# Autodesk Inventor assembly: CollectorAssembly
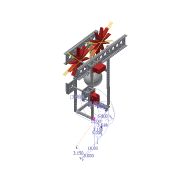
[picture p0: Inventor's stored thumbnail of the model, 180x180]
Saved by Autodesk Inventor 2018 (Build 220112000, 112)
## iProperties
Created: 2018-10-28
Part Number: CollectorAssembly
Document SubType Name: Assembly
Designer: ball
Author: ball
## Documents named in this file (18)
- C:\FTC\FTC8863CAD\2018Robot\CollectorAssembly.iam
- C:\FTC\FTC8863CAD\GoBilda\1103 Parts\1106-0035-0280.ipt
- C:\FTC\FTC8863CAD\GoBilda\1121 Parts\1121-0011-0288.ipt
- C:\FTC\FTC8863CAD\2018Robot\ServoWithPlateCoupler.iam
- C:\FTC\FTC8863CAD\GoBilda\1501 Parts\1501-0006-0240.ipt
- C:\FTC\FTC8863CAD\GoBilda\2905 Parts\2905-0006-0008 assembly.ipt
- C:\FTC\FTC8863CAD\GoBilda\1601 Parts\1601-0014-0006.ipt
- C:\FTC\FTC8863CAD\GoBilda\2101 Parts\2101-0006-0090.ipt
- C:\FTC\FTC8863CAD\Andymark\am-0619a+Entrapption+Star,+4.75+Diameter.ipt
- C:\FTC\FTC8863CAD\Andymark\am-2850+wiffle+base+Ball.ipt
- C:\FTC\FTC8863CAD\GoBilda\1103 Parts\1103-0011-0088.ipt
- C:\FTC\FTC8863CAD\GoBilda\1121 Parts\1121-0007-0192.ipt
- C:\FTC\FTC8863CAD\GoBilda\1106 Parts\1106-0010-0080.ipt
- C:\FTC\FTC8863CAD\RevRobotics\REV-31-1537.ipt
- C:\FTC\FTC8863CAD\GoBilda\1121 Parts\1121-0001-0048.ipt
- C:\FTC\FTC8863CAD\GoBilda\2101 Parts\2101-0006-0080.ipt
- C:\FTC\FTC8863CAD\GoBilda\1106 Parts\1106-0009-0072.ipt
- C:\FTC\FTC8863CAD\2018Robot\TransferChute.ipt
## Components (33 placed, 17 different names)
1. 1106-0035-0280:1 — Flush:1, Flush:2, Flush:4, Mate:62, Mate:63, Flush:5, Mate:70, Mate:101
2. 1106-0035-0280:2 — Flush:1, Flush:4, Mate:13, Mate:57, Mate:59, Mate:69, Mate:90, Mate:91, Mate:92
3. 1106-0035-0280:3 — Flush:2, Mate:58, Mate:69, Mate:74, Mate:75, Mate:93, Mate:95
4. 1106-0035-0280:4 — Mate:61, Flush:5, Mate:64, Mate:70, Mate:99, Mate:102, Mate:104
5. 1121-0011-0288:1 — Mate:13, Mate:22, Mate:23, Mate:24, Mate:25, Mate:26, Mate:27, Mate:37, Mate:38, Mate:68
6. ServoWithPlateCoupler:1 [sub-assembly] — Mate:15, Mate:17, Mate:19, Mate:21, Mate:22, Mate:27
7. 1501-0006-0240:2 — Mate:15, Mate:23
8. 1501-0006-0240:3 — Mate:19, Mate:25
9. 1501-0006-0240:4 — Mate:17, Mate:26
10. 1501-0006-0240:5 — Mate:21, Mate:24
11. 2905-0006-0008 assembly:1 — Mate:42, Mate:43
12. 2905-0006-0008 assembly:2 — Mate:44, Mate:45
13. 1601-0014-0006:1 — Mate:41, Mate:42, Mate:66
14. 1601-0014-0006:2 — Mate:37, Mate:38, Mate:40, Mate:44
15. 2101-0006-0090:1 — Mate:40, Mate:41, Mate:43, Mate:45, Mate:65, Mate:66, Mate:67
16. am-0619a+Entrapption+Star,+4.75+Diameter:1 — Mate:67, Mate:97
17. am-0619a+Entrapption+Star,+4.75+Diameter:2 — Mate:68, Mate:98
18. am-2850+wiffle+base+Ball:1
19. 1103-0011-0088:2 — Mate:61, Mate:62, Mate:63, Mate:78
20. 1103-0011-0088:3 — Mate:57, Mate:58, Mate:59, Mate:76, Mate:77, Flush:6
21. 1121-0007-0192:2 — Mate:64, Mate:65, Mate:74, Mate:75, Mate:97, Mate:98
22. 1106-0010-0080:1 — Mate:76, Mate:77, Flush:6, Mate:78
23. REV-31-1537:3 — Mate:99, Mate:103, Mate:104
24. ServoWithPlateCoupler:2 [sub-assembly] — Mate:88, Mate:89, Angle:1, Flush:8
25. 1501-0006-0240:6 — Mate:83, Mate:86
26. 1501-0006-0240:7 — Mate:84
27. 1501-0006-0240:8 — Mate:85
28. 1501-0006-0240:9 — Mate:88
29. 1121-0001-0048:1 — Mate:83, Mate:84, Mate:85, Mate:86, Mate:89, Angle:1, Mate:90, Mate:91, Mate:92, Mate:94, Flush:7
30. 1121-0001-0048:2 — Mate:93, Mate:94, Flush:7, Mate:95
31. 2101-0006-0080:2 — Flush:8
32. 1106-0009-0072:1 — Mate:101, Mate:102, Mate:103
33. TransferChute:1
## Relationships (69: Mate 61, Flush 7, Angle 1)
- Flush:1: 1106-0035-0280:1 ↔ 1106-0035-0280:2
- Flush:2: 1106-0035-0280:1 ↔ 1106-0035-0280:3
- Flush:4: 1106-0035-0280:1 ↔ 1106-0035-0280:2
- Mate:13: 1106-0035-0280:2 ↔ 1121-0011-0288:1
- Mate:15: ServoWithPlateCoupler:1 ↔ 1501-0006-0240:2
- Mate:17: ServoWithPlateCoupler:1 ↔ 1501-0006-0240:4
- Mate:19: ServoWithPlateCoupler:1 ↔ 1501-0006-0240:3
- Mate:21: ServoWithPlateCoupler:1 ↔ 1501-0006-0240:5
- Mate:22: 1121-0011-0288:1 ↔ ServoWithPlateCoupler:1
- Mate:23: 1121-0011-0288:1 ↔ 1501-0006-0240:2
- Mate:24: 1121-0011-0288:1 ↔ 1501-0006-0240:5
- Mate:25: 1121-0011-0288:1 ↔ 1501-0006-0240:3
- Mate:26: 1121-0011-0288:1 ↔ 1501-0006-0240:4
- Mate:27 (24 mm): 1121-0011-0288:1 ↔ ServoWithPlateCoupler:1
- Mate:37: 1121-0011-0288:1 ↔ 1601-0014-0006:2
- Mate:38: 1121-0011-0288:1 ↔ 1601-0014-0006:2
- Mate:40: 1601-0014-0006:2 ↔ 2101-0006-0090:1
- Mate:41: 1601-0014-0006:1 ↔ 2101-0006-0090:1
- Mate:42: 2905-0006-0008 assembly:1 ↔ 1601-0014-0006:1
- Mate:43: 2905-0006-0008 assembly:1 ↔ 2101-0006-0090:1
- Mate:44: 2905-0006-0008 assembly:2 ↔ 1601-0014-0006:2
- Mate:45: 2905-0006-0008 assembly:2 ↔ 2101-0006-0090:1
- Mate:57: 1106-0035-0280:2 ↔ 1103-0011-0088:3
- Mate:58: 1106-0035-0280:3 ↔ 1103-0011-0088:3
- Mate:59: 1106-0035-0280:2 ↔ 1103-0011-0088:3
- Mate:61: 1106-0035-0280:4 ↔ 1103-0011-0088:2
- Mate:62: 1106-0035-0280:1 ↔ 1103-0011-0088:2
- Mate:63: 1106-0035-0280:1 ↔ 1103-0011-0088:2
- Flush:5: 1106-0035-0280:1 ↔ 1106-0035-0280:4
- Mate:64: 1106-0035-0280:4 ↔ 1121-0007-0192:2
- Mate:65: 2101-0006-0090:1 ↔ 1121-0007-0192:2
- Mate:66: 1601-0014-0006:1 ↔ 2101-0006-0090:1
- Mate:67: 2101-0006-0090:1 ↔ am-0619a+Entrapption+Star,+4.75+Diameter:1
- Mate:68: 1121-0011-0288:1 ↔ am-0619a+Entrapption+Star,+4.75+Diameter:2
- Mate:69: 1106-0035-0280:2 ↔ 1106-0035-0280:3
- Mate:70: 1106-0035-0280:1 ↔ 1106-0035-0280:4
- Mate:74: 1106-0035-0280:3 ↔ 1121-0007-0192:2
- Mate:75: 1106-0035-0280:3 ↔ 1121-0007-0192:2
- Mate:76: 1103-0011-0088:3 ↔ 1106-0010-0080:1
- Mate:77: 1103-0011-0088:3 ↔ 1106-0010-0080:1
- Flush:6: 1103-0011-0088:3 ↔ 1106-0010-0080:1
- Mate:78: 1103-0011-0088:2 ↔ 1106-0010-0080:1
- [Mate]: ServoWithPlateCoupler:2 ↔ 1501-0006-0240:6
- [Mate]: ServoWithPlateCoupler:2 ↔ 1501-0006-0240:8
- [Mate]: ServoWithPlateCoupler:2 ↔ 1501-0006-0240:7
- [Mate]: ServoWithPlateCoupler:2 ↔ 1501-0006-0240:9
- Mate:83: 1501-0006-0240:6 ↔ 1121-0001-0048:1
- Mate:84: 1501-0006-0240:7 ↔ 1121-0001-0048:1
- Mate:85: 1501-0006-0240:8 ↔ 1121-0001-0048:1
- Mate:86: 1501-0006-0240:6 ↔ 1121-0001-0048:1
- Mate:88: ServoWithPlateCoupler:2 ↔ 1501-0006-0240:9
- Mate:89: ServoWithPlateCoupler:2 ↔ 1121-0001-0048:1
- Angle:1 (0 deg): ServoWithPlateCoupler:2 ↔ 1121-0001-0048:1
- Mate:90: 1106-0035-0280:2 ↔ 1121-0001-0048:1
- Mate:91: 1106-0035-0280:2 ↔ 1121-0001-0048:1
- Mate:92: 1106-0035-0280:2 ↔ 1121-0001-0048:1
- Mate:93: 1106-0035-0280:3 ↔ 1121-0001-0048:2
- Mate:94: 1121-0001-0048:1 ↔ 1121-0001-0048:2
- Flush:7: 1121-0001-0048:1 ↔ 1121-0001-0048:2
- Mate:95: 1106-0035-0280:3 ↔ 1121-0001-0048:2
- [Mate]: 1121-0001-0048:2 ↔ 2101-0006-0080:2
- Flush:8: ServoWithPlateCoupler:2 ↔ 2101-0006-0080:2
- Mate:97 (33.3375 mm): am-0619a+Entrapption+Star,+4.75+Diameter:1 ↔ 1121-0007-0192:2
- Mate:98 (19.05 mm): am-0619a+Entrapption+Star,+4.75+Diameter:2 ↔ 1121-0007-0192:2
- Mate:99: 1106-0035-0280:4 ↔ REV-31-1537:3
- Mate:101: 1106-0035-0280:1 ↔ 1106-0009-0072:1
- Mate:102: 1106-0035-0280:4 ↔ 1106-0009-0072:1
- Mate:103: REV-31-1537:3 ↔ 1106-0009-0072:1
- Mate:104 (16.2814 mm): 1106-0035-0280:4 ↔ REV-31-1537:3
## Named parameters: d97_d28 = 0 mm, d98_d30 = 0 mm, d99_d32 = 0 mm, d100_d34 = 0 mm
